# Autodesk Inventor assembly: Drivebase
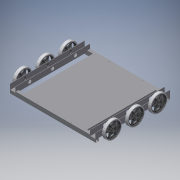
[picture p0: Inventor's stored thumbnail of the model, 180x180]
Saved by Autodesk Inventor 2018 (Build 220112000, 112)
## iProperties
Created: 2018-06-29
Part Number: Drivebase
Document SubType Name: Assembly
Designer: s-2512711
Author: s-2512711
## Documents named in this file (5)
- \\studenthome\students\S-2512711\Inventor\Drivebase.iam
- \\studenthome\students\S-2512711\Inventor\u-channel.ipt
- \\studenthome\students\S-2512711\Inventor\1x1.ipt
- C:\Users\s-2512711\Downloads\2008-FIRST-Wheel.iam
- \\studenthome\students\S-2512711\Inventor\pan.ipt
## Components (11 placed, 4 different names)
1. u-channel:1 — Mate:7, Mate:8, Mate:9, Mate:10, Mate:11, Rotation:1, Mate:12, Mate:13, Rotation:2, Mate:14, Mate:15, Rotation:3
2. u-channel:2 — Mate:1, Mate:2, Mate:3, Mate:4, Mate:5, Mate:6, Mate:16, Mate:17, Rotation:4, Mate:18, Mate:19, Rotation:5, Mate:20, Mate:21, Rotation:6, Mate:24
3. 1x1:1 — Mate:4, Mate:5, Mate:6, Mate:7, Mate:8, Mate:9, Mate:22, Mate:23
4. 1x1:2 — Mate:1, Mate:2, Mate:3
5. 2008-FIRST-Wheel:1 [sub-assembly] — Mate:20, Mate:21, Rotation:6
6. 2008-FIRST-Wheel:2 [sub-assembly] — Mate:16, Mate:17, Rotation:4
7. 2008-FIRST-Wheel:3 [sub-assembly] — Mate:18, Mate:19, Rotation:5
8. 2008-FIRST-Wheel:4 [sub-assembly] — Mate:10, Mate:11, Rotation:1
9. 2008-FIRST-Wheel:5 [sub-assembly] — Mate:12, Mate:13, Rotation:2
10. 2008-FIRST-Wheel:6 [sub-assembly] — Mate:14, Mate:15, Rotation:3
11. pan:1 — Mate:22, Mate:23, Mate:24
## Relationships (30: Mate 24, RelateRotation 6)
- Mate:1: u-channel:2 ↔ 1x1:2
- Mate:2: u-channel:2 ↔ 1x1:2
- Mate:3: u-channel:2 ↔ 1x1:2
- Mate:4: u-channel:2 ↔ 1x1:1
- Mate:5: u-channel:2 ↔ 1x1:1
- Mate:6: u-channel:2 ↔ 1x1:1
- Mate:7: u-channel:1 ↔ 1x1:1
- Mate:8: u-channel:1 ↔ 1x1:1
- Mate:9: u-channel:1 ↔ 1x1:1
- Mate:10: u-channel:1 ↔ 2008-FIRST-Wheel:4
- Mate:11: u-channel:1 ↔ 2008-FIRST-Wheel:4
- Rotation:1 [RelateRotation] (1 ul): u-channel:1 ↔ 2008-FIRST-Wheel:4
- Mate:12: u-channel:1 ↔ 2008-FIRST-Wheel:5
- Mate:13: u-channel:1 ↔ 2008-FIRST-Wheel:5
- Rotation:2 [RelateRotation] (1 ul): u-channel:1 ↔ 2008-FIRST-Wheel:5
- Mate:14: u-channel:1 ↔ 2008-FIRST-Wheel:6
- Mate:15: u-channel:1 ↔ 2008-FIRST-Wheel:6
- Rotation:3 [RelateRotation] (1 ul): u-channel:1 ↔ 2008-FIRST-Wheel:6
- Mate:16: u-channel:2 ↔ 2008-FIRST-Wheel:2
- Mate:17: u-channel:2 ↔ 2008-FIRST-Wheel:2
- Rotation:4 [RelateRotation] (1 ul): u-channel:2 ↔ 2008-FIRST-Wheel:2
- Mate:18: u-channel:2 ↔ 2008-FIRST-Wheel:3
- Mate:19: u-channel:2 ↔ 2008-FIRST-Wheel:3
- Rotation:5 [RelateRotation] (1 ul): u-channel:2 ↔ 2008-FIRST-Wheel:3
- Mate:20: u-channel:2 ↔ 2008-FIRST-Wheel:1
- Mate:21: u-channel:2 ↔ 2008-FIRST-Wheel:1
- Rotation:6 [RelateRotation] (1 ul): u-channel:2 ↔ 2008-FIRST-Wheel:1
- Mate:22: 1x1:1 ↔ pan:1
- Mate:23: 1x1:1 ↔ pan:1
- Mate:24: u-channel:2 ↔ pan:1
